# Autodesk Inventor assembly: noze-cone
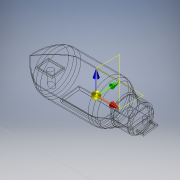
[picture p0: Inventor's stored thumbnail of the model, 180x180]
Saved by Autodesk Inventor 2017 (Build 210142000, 142)
## iProperties
Created: 2020-06-18
Part Number: noze-cone
Document SubType Name: Assembly
Designer: HAYNIE R&D
Author: HAYNIE R&D
## Documents named in this file (3)
- C:\Users\HAYNIE\source\repos\telemetry\3d-models\noze-cone.iam
- C:\Users\HAYNIE\source\repos\telemetry\3d-models\noze-cone-side-1.ipt
- C:\Users\HAYNIE\source\repos\telemetry\3d-models\noze-cone-side-2.ipt
## Components (2 placed, 2 different names)
1. noze-cone-side-1:1 — Cylindrical:1
2. noze-cone-side-2:1 — Cylindrical:1
## Relationships (1: CylindricalJoint 1)
- Cylindrical:1: noze-cone-side-1:1 ↔ noze-cone-side-2:1
